# Autodesk Inventor assembly: Portamarcadorv2
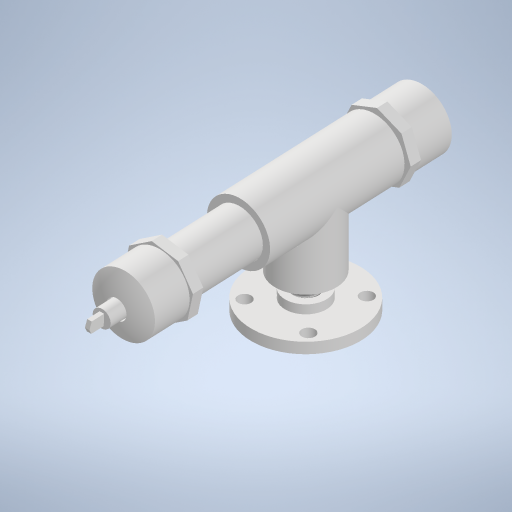
[picture p0: Inventor's stored thumbnail of the model, 512x512]
Saved by Autodesk Inventor 2023.1 (Build 271208000, 208)
## iProperties
Created: 2022-08-28
Part Number: Portamarcadorv2
Document SubType Name: Assembly
Designer: Daniel Peña
Author: Daniel Peña
## Documents named in this file (8)
- C:\Users\danie_p\Documents\Inventor\Lab1Robotica\Portamarcadorv2.iam
- C:\Users\danie_p\Documents\Inventor\Lab1Robotica\TuboL.ipt
- C:\Users\danie_p\Documents\Inventor\Lab1Robotica\TapaPVC.ipt
- C:\Users\danie_p\Documents\Inventor\Lab1Robotica\T_PVC.ipt
- C:\Users\danie_p\Documents\Inventor\Lab1Robotica\TuboC.ipt
- C:\Users\danie_p\Documents\Inventor\Lab1Robotica\PortaMandril.ipt
- C:\Users\danie_p\Documents\Inventor\Lab1Robotica\Resorte.ipt
- C:\Users\danie_p\Documents\Inventor\Lab1Robotica\Pelikan426.ipt
## Components (9 placed, 7 different names)
1. TuboL:1 — Insert:3, Insert:4
2. TapaPVC:1 — Insert:4, Insert:8
3. T_PVC:1 — Insert:2, Insert:3, Insert:9
4. TuboC:1 — Insert:1, Insert:2
5. TapaPVC:2 — Insert:1, Insert:7
6. PortaMandril:1 — Insert:9
7. Resorte:1 — Insert:6
8. Resorte:2 — Insert:6, Insert:7
9. Pelikan426:1 — Flush:1, Insert:8
## Relationships (9: Insert 8, Flush 1)
- Insert:1: TuboC:1 ↔ TapaPVC:2
- Insert:2: T_PVC:1 ↔ TuboC:1
- Insert:3: TuboL:1 ↔ T_PVC:1
- Insert:4: TuboL:1 ↔ TapaPVC:1
- Insert:6: Resorte:1 ↔ Resorte:2
- Insert:7: TapaPVC:2 ↔ Resorte:2
- Flush:1: Pelikan426:1
- Insert:8: TapaPVC:1 ↔ Pelikan426:1
- Insert:9 (11 mm): T_PVC:1 ↔ PortaMandril:1
